# Autodesk Inventor assembly: Picker Tool
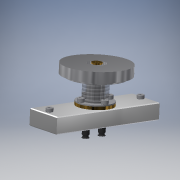
[picture p0: Inventor's stored thumbnail of the model, 180x180]
Saved by Autodesk Inventor 2019.4 (Build 234330000, 330)
## iProperties
Created: 2021-01-08
Part Number: Picker Tool
Document SubType Name: Assembly
Designer: caleb
Author: caleb
## Documents named in this file (6)
- C:\Users\cfang\Desktop\nebraska-silicon-lab\CAD\ETL\Module Assembly\Picker Tool\Picker Tool.iam
- C:\Users\cfang\Desktop\nebraska-silicon-lab\CAD\ETL\Module Assembly\Picker Tool\Picker Base.ipt
- C:\Users\cfang\Desktop\nebraska-silicon-lab\CAD\ETL\Module Assembly\Picker Tool\Bellows Assembly.iam
- C:\Users\cfang\Desktop\nebraska-silicon-lab\CAD\ETL\Module Assembly\Picker Tool\Platform Assembly.iam
- C:\Users\cfang\Desktop\nebraska-silicon-lab\CAD\ETL\Module Assembly\Picker Tool\91290A119_BLACK-OXIDE CLASS 12.9 SOCKET HEAD CAP SCREW.ipt
- C:\Users\cfang\Desktop\nebraska-silicon-lab\CAD\ETL\Module Assembly\Picker Tool\Spool Assembly.iam
## Components (8 placed, 5 different names)
1. Picker Base:1 — Insert:2, Rotational:1, Cylindrical:1
2. Bellows Assembly:1 [sub-assembly] — Insert:2, Rotational:1, Insert:3, Insert:4, Insert:5, Insert:6, Insert:7
3. Platform Assembly:1 [sub-assembly] — Rotational:2
4. 91290A119_BLACK-OXIDE CLASS 12.9 SOCKET HEAD CAP SCREW:1 — Insert:5
5. 91290A119_BLACK-OXIDE CLASS 12.9 SOCKET HEAD CAP SCREW:2 — Insert:4
6. 91290A119_BLACK-OXIDE CLASS 12.9 SOCKET HEAD CAP SCREW:3 — Insert:6
7. 91290A119_BLACK-OXIDE CLASS 12.9 SOCKET HEAD CAP SCREW:4 — Insert:7
8. Spool Assembly:1 [sub-assembly] — Cylindrical:1, Insert:3, Rotational:2
## Relationships (9: Insert 6, RevoluteJoint 2, CylindricalJoint 1)
- Insert:2: Picker Base:1 ↔ Bellows Assembly:1
- Rotational:1 [RevoluteJoint]: Picker Base:1 ↔ Bellows Assembly:1
- Cylindrical:1: Picker Base:1 ↔ Spool Assembly:1
- Insert:3: Bellows Assembly:1 ↔ Spool Assembly:1
- Rotational:2 [RevoluteJoint]: Platform Assembly:1 ↔ Spool Assembly:1
- Insert:4: Bellows Assembly:1 ↔ 91290A119_BLACK-OXIDE CLASS 12.9 SOCKET HEAD CAP SCREW:2
- Insert:5: Bellows Assembly:1 ↔ 91290A119_BLACK-OXIDE CLASS 12.9 SOCKET HEAD CAP SCREW:1
- Insert:6: Bellows Assembly:1 ↔ 91290A119_BLACK-OXIDE CLASS 12.9 SOCKET HEAD CAP SCREW:3
- Insert:7: Bellows Assembly:1 ↔ 91290A119_BLACK-OXIDE CLASS 12.9 SOCKET HEAD CAP SCREW:4
